# Autodesk Inventor assembly: ENSAMBLE_TOTAL
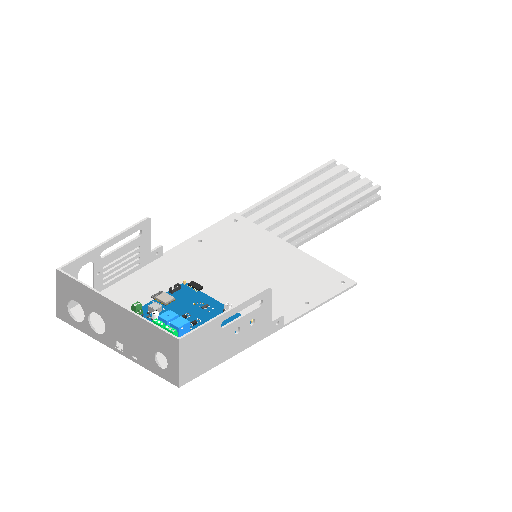
[picture p0: Inventor's stored thumbnail of the model, 512x512]
Saved by Autodesk Inventor 2025 (Build 290162000, 162)
## iProperties
Created: 2026-02-14
Part Number: ENSAMBLE_TOTAL
Document SubType Name: Assembly
Designer: HP
Author: HP
## Documents named in this file (5)
- C:\Users\HP\Desktop\TESIS 2\TFC2_20212123_MHinojosa\TFC2-20212123-HW\CAD\PLANOS\ENSAMBLE_TOTAL.iam
- C:\Users\HP\Desktop\TESIS 2\TFC2_20212123_MHinojosa\TFC2-20212123-HW\CAD\3D_PCB10_2026-02-04\3D_PCB10_2026-02-04.ipt
- C:\Users\HP\Desktop\TESIS 2\TFC2_20212123_MHinojosa\TFC2-20212123-HW\CAD\Chasis\Chasis_CONTROL.ipt
- C:\Users\HP\Desktop\TESIS 2\TFC2_20212123_MHinojosa\TFC2-20212123-HW\CAD\M3 x 10 Brass Standoff_\M3 x 10 Brass Standoff_.ipt
- C:\Users\HP\Desktop\TESIS 2\TFC2_20212123_MHinojosa\TFC2-20212123-HW\CAD\Profiles\Profiles.ipt
## Components (7 placed, 4 different names)
1. Chasis_CONTROL:1 — Nivelación:1, Nivelación:2, Nivelación:3, Coincidencia:1, Coincidencia:2, Coincidencia:3, Coincidencia:4, Coincidencia:5
2. M3 x 10 Brass Standoff_:1 — Nivelación:4, Coincidencia:5, Coincidencia:6
3. M3 x 10 Brass Standoff_:2 — Nivelación:4, Nivelación:5, Nivelación:6, Coincidencia:4
4. M3 x 10 Brass Standoff_:3 — Nivelación:5, Coincidencia:3, Coincidencia:8
5. M3 x 10 Brass Standoff_:4 — Nivelación:6, Coincidencia:1, Coincidencia:2, Coincidencia:7
6. 3D_PCB10_2026-02-04:1 — Coincidencia:6, Coincidencia:7, Coincidencia:8
7. Profiles:1
## Relationships (14: Mate 8, Flush 6)
- Nivelación:1 [Flush]: Chasis_CONTROL:1
- Nivelación:2 [Flush]: Chasis_CONTROL:1
- Nivelación:3 [Flush]: Chasis_CONTROL:1
- Nivelación:4 [Flush]: M3 x 10 Brass Standoff_:1 ↔ M3 x 10 Brass Standoff_:2
- Nivelación:5 [Flush]: M3 x 10 Brass Standoff_:2 ↔ M3 x 10 Brass Standoff_:3
- Nivelación:6 [Flush]: M3 x 10 Brass Standoff_:2 ↔ M3 x 10 Brass Standoff_:4
- Coincidencia:1 [Mate]: Chasis_CONTROL:1 ↔ M3 x 10 Brass Standoff_:4
- Coincidencia:2 [Mate]: Chasis_CONTROL:1 ↔ M3 x 10 Brass Standoff_:4
- Coincidencia:3 [Mate]: Chasis_CONTROL:1 ↔ M3 x 10 Brass Standoff_:3
- Coincidencia:4 [Mate]: Chasis_CONTROL:1 ↔ M3 x 10 Brass Standoff_:2
- Coincidencia:5 [Mate]: Chasis_CONTROL:1 ↔ M3 x 10 Brass Standoff_:1
- Coincidencia:6 [Mate]: M3 x 10 Brass Standoff_:1 ↔ 3D_PCB10_2026-02-04:1
- Coincidencia:7 [Mate]: M3 x 10 Brass Standoff_:4 ↔ 3D_PCB10_2026-02-04:1
- Coincidencia:8 [Mate]: M3 x 10 Brass Standoff_:3 ↔ 3D_PCB10_2026-02-04:1
